# Autodesk Inventor assembly: Arm
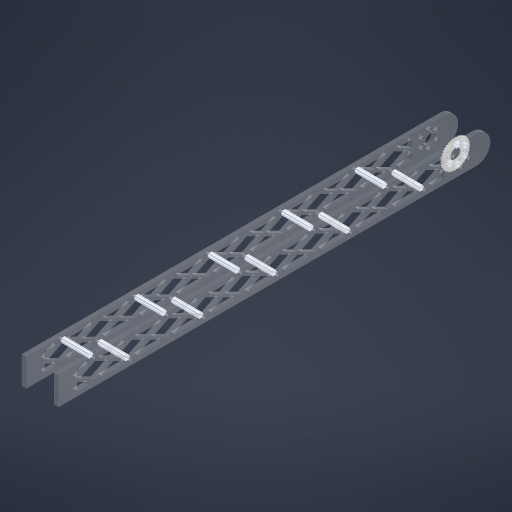
[picture p0: Inventor's stored thumbnail of the model, 512x512]
Saved by Autodesk Inventor 2023 (Build 270158000, 158)
## iProperties
Created: 2023-01-21
Part Number: Arm
Document SubType Name: Assembly
Designer: Terrence
Mass: 1817.68 g
Surface Area: 4767.56 cm^2
Volume: 1413.39 cm^3
Density: 1.28604 g/cm^3
Author: Terrence
## Documents named in this file (5)
- C:\Users\Terrence\Documents\FRC Long\Arm\Arm.iam
- C:\Users\Terrence\Documents\FRC Long\Arm\Solid1.ipt
- C:\Users\Terrence\Documents\FRC Long\Arm\am-churro 500 churro tube1.ipt
- C:\Users\Terrence\Documents\FRC Long\Arm\am-0661 38T 25 Chain Bearing Bore Sprocket.ipt
- C:\Users\Terrence\Documents\FRC Long\Newvator\am-churro 500 churro tube - Copy.ipt
## Components (18 placed, 4 different names)
1. Solid1:1 — Insert:1, Insert:2, Insert:3, Insert:4, Insert:5, Insert:6, Insert:7, Insert:8, Insert:9, Insert:10
2. am-churro 500 churro tube1:1 — Insert:1, Insert:11
3. am-0661 38T 25 Chain Bearing Bore Sprocket:1 — Insert:18
4. am-churro 500 churro tube1:2 — Insert:2, Insert:12
5. am-churro 500 churro tube1:3 — Insert:3
6. am-churro 500 churro tube1:4 — Insert:4
7. am-churro 500 churro tube1:5 — Insert:6
8. am-churro 500 churro tube1:6 — Insert:5
9. am-churro 500 churro tube1:7 — Insert:9
10. am-churro 500 churro tube1:8 — Insert:10
11. am-churro 500 churro tube1:9 — Insert:8
12. am-churro 500 churro tube1:10 — Insert:7
13. Solid1:2 — Insert:11, Insert:12, Insert:13, Insert:14, Insert:15, Insert:16, Insert:17, Insert:18
14. am-churro 500 churro tube - Copy:1 — Insert:13
15. am-churro 500 churro tube - Copy:2 — Insert:17
16. am-churro 500 churro tube - Copy:3 — Insert:16
17. am-churro 500 churro tube - Copy:4 — Insert:14
18. am-churro 500 churro tube - Copy:5 — Insert:15
## Relationships (18: Insert 18)
- Insert:1: Solid1:1 ↔ am-churro 500 churro tube1:1
- Insert:2: Solid1:1 ↔ am-churro 500 churro tube1:2
- Insert:3: Solid1:1 ↔ am-churro 500 churro tube1:3
- Insert:4: Solid1:1 ↔ am-churro 500 churro tube1:4
- Insert:5: Solid1:1 ↔ am-churro 500 churro tube1:6
- Insert:6: Solid1:1 ↔ am-churro 500 churro tube1:5
- Insert:7: Solid1:1 ↔ am-churro 500 churro tube1:10
- Insert:8: Solid1:1 ↔ am-churro 500 churro tube1:9
- Insert:9: Solid1:1 ↔ am-churro 500 churro tube1:7
- Insert:10: Solid1:1 ↔ am-churro 500 churro tube1:8
- Insert:11: am-churro 500 churro tube1:1 ↔ Solid1:2
- Insert:12: am-churro 500 churro tube1:2 ↔ Solid1:2
- Insert:13: Solid1:2 ↔ am-churro 500 churro tube - Copy:1
- Insert:14: Solid1:2 ↔ am-churro 500 churro tube - Copy:4
- Insert:15: Solid1:2 ↔ am-churro 500 churro tube - Copy:5
- Insert:16: Solid1:2 ↔ am-churro 500 churro tube - Copy:3
- Insert:17: Solid1:2 ↔ am-churro 500 churro tube - Copy:2
- Insert:18 (6.35 mm): am-0661 38T 25 Chain Bearing Bore Sprocket:1 ↔ Solid1:2
